# Autodesk Inventor assembly: SLIPRING_SRG-1-6G
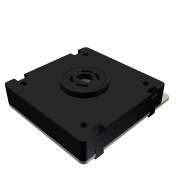
[picture p0: Inventor's stored thumbnail of the model, 180x180]
Saved by Autodesk Inventor 2011 SP1 (Build 150282100, 282)
## iProperties
Created: 2012-05-23
Part Number: SLIPRING_SRG-1-6G
Document SubType Name: Assembly
Designer: arihon
Author: arihon
## Documents named in this file (4)
- C:\Users\arihon\Dropbox\Inventor\walkPivot\walkingCDGA\SLIPRING_SRG-1-6G.iam
- C:\Users\arihon\Dropbox\Inventor\walkPivot\walkingCDGA\SLIPRING_SRG-1-6G.ipt
- C:\Users\arihon\Dropbox\Inventor\walkPivot\walkingCDGA\SLIPRING_SRG-1-6G_.ipt
- C:\Users\arihon\Dropbox\Inventor\walkPivot\walkingCDGA\SLIPRING_SRG-1-6G_シャフト.ipt
## Components (3 placed, 3 different names)
1. SLIPRING_SRG-1-6G:1 — 挿入:1, 挿入:2, 挿入:3
2. SLIPRING_SRG-1-6G_:1 — 挿入:1, 挿入:2
3. SLIPRING_SRG-1-6G_シャフト:1 — 挿入:3
## Relationships (3: Insert 3)
- 挿入:1 [Insert]: SLIPRING_SRG-1-6G:1 ↔ SLIPRING_SRG-1-6G_:1
- 挿入:2 [Insert]: SLIPRING_SRG-1-6G:1 ↔ SLIPRING_SRG-1-6G_:1
- 挿入:3 [Insert]: SLIPRING_SRG-1-6G:1 ↔ SLIPRING_SRG-1-6G_シャフト:1
